# Autodesk Inventor assembly: Montagem Motor
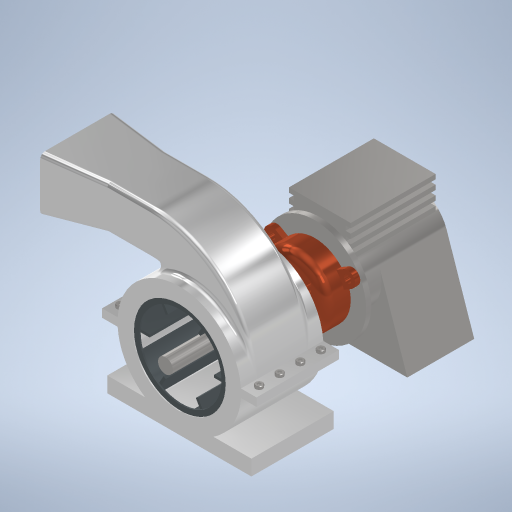
[picture p0: Inventor's stored thumbnail of the model, 512x512]
Saved by Autodesk Inventor 2023.2 (Build 272271000, 271)
## iProperties
Created: 2022-12-18
Part Number: Montagem Motor
Document SubType Name: Assembly
Designer: coqui
Author: coqui
## Documents named in this file (8)
- D:\Felipe Coquito\OneDrive\Documents\Inventor\Inventor - curso\Montagem\Montagem Motor.iam
- D:\Felipe Coquito\OneDrive\Documents\Inventor\Inventor - curso\Motor Industrial\Carcaça Inferior do Motor Industiral.ipt
- D:\Felipe Coquito\OneDrive\Documents\Inventor\Inventor - curso\Motor Industrial\Cilindro do Motor Industrial.ipt
- D:\Felipe Coquito\OneDrive\Documents\Inventor\Inventor - curso\Motor Industrial\Carcaça Superior do Motor Industrial.ipt
- D:\Felipe Coquito\OneDrive\Documents\Inventor\Inventor - curso\Motor Industrial\Disco do Motor Industrial.ipt
- D:\Felipe Coquito\OneDrive\Documents\Inventor\Inventor - curso\Motor Industrial\Base do Motor Industrial.ipt
- D:\Felipe Coquito\OneDrive\Documents\Inventor\Inventor - curso\Motor Industrial\Eixo do Motor Industrial.ipt
- D:\Felipe Coquito\OneDrive\Documents\Inventor\Content Center Files\R2023\en-US\DIN 6912\DIN 6912 - M4 x 10.ipt
## Components (14 placed, 7 different names)
1. Carcaça Inferior do Motor Industiral:1 — Mate:1, Mate:2, Mate:3, Mate:9
2. Cilindro do Motor Industrial:1 — Mate:1, Mate:2, Mate:4, Mate:5
3. Carcaça Superior do Motor Industrial:1 — Mate:3, Mate:9, Mate:12, Mate:13
4. Disco do Motor Industrial:1 — Mate:4, Mate:5, Mate:6, Mate:7, Mate:8
5. Base do Motor Industrial:1 — Mate:6, Mate:7, Mate:8, Mate:10, Mate:11
6. Eixo do Motor Industrial:1 — Mate:10, Mate:11
7. DIN 6912 M4 x 10:1 — Mate:12, Mate:13
8. DIN 6912 M4 x 10:2
9. DIN 6912 M4 x 10:3
10. DIN 6912 M4 x 10:4
11. DIN 6912 M4 x 10:5
12. DIN 6912 M4 x 10:6
13. DIN 6912 M4 x 10:7
14. DIN 6912 M4 x 10:8
## Component patterns: (8 elements, first: DIN 6912 M4 x 10:1)
## Relationships (13: Mate 13)
- Mate:1: Carcaça Inferior do Motor Industiral:1 ↔ Cilindro do Motor Industrial:1
- Mate:2: Carcaça Inferior do Motor Industiral:1 ↔ Cilindro do Motor Industrial:1
- Mate:3: Carcaça Inferior do Motor Industiral:1 ↔ Carcaça Superior do Motor Industrial:1
- Mate:4: Cilindro do Motor Industrial:1 ↔ Disco do Motor Industrial:1
- Mate:5: Cilindro do Motor Industrial:1 ↔ Disco do Motor Industrial:1
- Mate:6: Disco do Motor Industrial:1 ↔ Base do Motor Industrial:1
- Mate:7: Disco do Motor Industrial:1 ↔ Base do Motor Industrial:1
- Mate:8: Disco do Motor Industrial:1 ↔ Base do Motor Industrial:1
- Mate:9: Carcaça Inferior do Motor Industiral:1 ↔ Carcaça Superior do Motor Industrial:1
- Mate:10: Base do Motor Industrial:1 ↔ Eixo do Motor Industrial:1
- Mate:11: Base do Motor Industrial:1 ↔ Eixo do Motor Industrial:1
- Mate:12: Carcaça Superior do Motor Industrial:1 ↔ DIN 6912 M4 x 10:1
- Mate:13: Carcaça Superior do Motor Industrial:1 ↔ DIN 6912 M4 x 10:1
